# Autodesk Inventor assembly: Cyclo_final
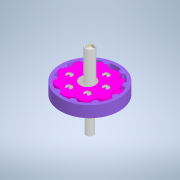
[picture p0: Inventor's stored thumbnail of the model, 180x180]
Saved by Autodesk Inventor 2022 (Build 260153000, 153)
## iProperties
Created: 2021-07-18
Part Number: Cyclo_final
Document SubType Name: Assembly
Designer: Madhav
Author: Madhav
## Documents named in this file (7)
- D:\MTAB\final\Cyclo_final.iam
- D:\MTAB\final\ring.ipt
- D:\MTAB\final\disc.ipt
- D:\MTAB\final\input_shaft.ipt
- D:\MTAB\final\Output_shaft.ipt
- C:\Users\Madhav\Downloads\TS4603N1000.ipt
- D:\MTAB\final\mounted_bearing.ipt
## Components (7 placed, 6 different names)
1. ring:1 — Rotational:4
2. disc:1 — Rotational:1
3. input_shaft:1 — Rotational:1, Rotational:3, Rotational:5, Rigid:1
4. disc:2 — Rotational:3
5. Output_shaft:1 — Rotational:4, Rotational:5
6. TS4603N1000:1 — Rigid:1
7. mounted_bearing:1
## Relationships (5: RevoluteJoint 4, WeldJoint 1)
- Rotational:1 [RevoluteJoint]: disc:1 ↔ input_shaft:1
- Rotational:3 [RevoluteJoint]: input_shaft:1 ↔ disc:2
- Rotational:4 [RevoluteJoint]: ring:1 ↔ Output_shaft:1
- Rotational:5 [RevoluteJoint] (5 mm): input_shaft:1 ↔ Output_shaft:1
- Rigid:1 [WeldJoint]: input_shaft:1 ↔ TS4603N1000:1
